# Autodesk Inventor assembly: Assembly1
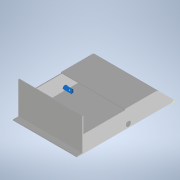
[picture p0: Inventor's stored thumbnail of the model, 180x180]
Saved by Autodesk Inventor 2022 (Build 260153000, 153)
## iProperties
Created: 2021-12-09
Part Number: Assembly1
Document SubType Name: Assembly
Designer: keemi
Author: keemi
## Documents named in this file (7)
- C:\Users\keemi\OneDrive\Documents\Inventor\Auto\eriks fiasco\Assembly1.iam
- C:\Users\keemi\OneDrive\Documents\Inventor\Auto\eriks fiasco\Part7.ipt
- C:\Users\keemi\OneDrive\Documents\Inventor\Auto\eriks fiasco\Part6.ipt
- C:\Users\keemi\OneDrive\Documents\Inventor\Auto\ir_sensor-1.snapshot.1\IR sensor.ipt
- C:\Users\keemi\OneDrive\Documents\Inventor\Auto\eriks fiasco\Part10.ipt
- C:\Users\keemi\OneDrive\Documents\Inventor\Auto\eriks fiasco\Part11.ipt
- C:\Users\keemi\OneDrive\Documents\Inventor\Auto\eriks fiasco\Part12.ipt
## Components (7 placed, 6 different names)
1. Part7:1 — Mate:2, Flush:2, Mate:6, Flush:3, Flush:4
2. Part6:1 — Mate:1, Mate:2, Flush:1, Flush:2, Mate:9, Mate:10
3. Part7:2 — Mate:1, Flush:1, Mate:5, Mate:7, Mate:8, Mate:11, Mate:13, Flush:5
4. IR sensor:1 — Mate:5, Mate:11
5. Part10:1 — Mate:6, Flush:3, Mate:7, Mate:10, Mate:14
6. Part11:1 — Mate:8, Flush:4, Mate:9
7. Part12:1 — Mate:13, Flush:5, Mate:14
## Relationships (16: Mate 11, Flush 5)
- Mate:1: Part6:1 ↔ Part7:2
- Mate:2: Part7:1 ↔ Part6:1
- Flush:1: Part6:1 ↔ Part7:2
- Flush:2: Part7:1 ↔ Part6:1
- Mate:5: Part7:2 ↔ IR sensor:1
- Mate:6: Part7:1 ↔ Part10:1
- Flush:3: Part7:1 ↔ Part10:1
- Mate:7: Part7:2 ↔ Part10:1
- Mate:8: Part7:2 ↔ Part11:1
- Flush:4: Part7:1 ↔ Part11:1
- Mate:9: Part6:1 ↔ Part11:1
- Mate:10: Part6:1 ↔ Part10:1
- Mate:11: Part7:2 ↔ IR sensor:1
- Mate:13: Part7:2 ↔ Part12:1
- Flush:5: Part7:2 ↔ Part12:1
- Mate:14: Part10:1 ↔ Part12:1
